# Autodesk Inventor assembly: full_rack
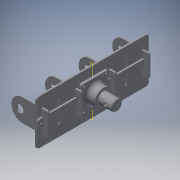
[picture p0: Inventor's stored thumbnail of the model, 180x180]
Saved by Autodesk Inventor 2016 (Build 200138000, 138)
## iProperties
Created: 2018-10-08
Part Number: full_rack
Document SubType Name: Assembly
Designer: andrew
Author: andrew
## Documents named in this file (6)
- C:\Users\andre\OneDrive\Uni_Work\Bench_corrosion_motor\Sample_rack\full_rack.iam
- C:\Users\andre\OneDrive\Uni_Work\Bench_corrosion_motor\Sample_rack\sample_mount.ipt
- C:\Users\andre\OneDrive\Uni_Work\Bench_corrosion_motor\Sample_rack\mounting_plate.ipt
- C:\Users\andre\OneDrive\Uni_Work\Bench_corrosion_motor\Sample_rack\pin.ipt
- C:\Users\andre\OneDrive\Uni_Work\Bench_corrosion_motor\Sample_rack\adaptor.ipt
- C:\Users\andre\OneDrive\Uni_Work\Bench_corrosion_motor\Sample_rack\full_rack\Design Accelerator\Bolted Connection1.iam
## Components (8 placed, 5 different names)
1. mounting_plate:1 — Rigid:1, Rotational:1, Rotational:2
2. pin:1 — Rotational:1, Mate:1
3. adaptor:1 — Rotational:2
4. Bolted Connection:1 [sub-assembly] — Mate:1
5. sample_mount:1 — Rigid:1
6. sample_mount:2
7. sample_mount:3
8. sample_mount:4
## Component patterns: (4 elements, first: sample_mount:1)
## Relationships (4: RevoluteJoint 2, WeldJoint 1, Mate 1)
- Rigid:1 [WeldJoint]: mounting_plate:1 ↔ sample_mount:1
- Rotational:1 [RevoluteJoint]: mounting_plate:1 ↔ pin:1
- Rotational:2 [RevoluteJoint]: mounting_plate:1 ↔ adaptor:1
- Mate:1: pin:1 ↔ Bolted Connection:1
